# Autodesk Inventor assembly: EFOI-10
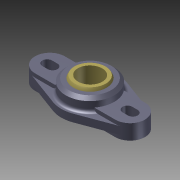
[picture p0: Inventor's stored thumbnail of the model, 180x180]
Saved by Autodesk Inventor 2011 (Build 150239000, 239)
## iProperties
Category: Plastic Bearings
Created: 2008-11-25
Part Number: EFOI-10
Document SubType Name: Assembly
Project: FIRST
Catalog Web Link: http://www.igus.com/pdf/igubal_flange.pdf
Description: Flanged spherical bearing
Vendor: igus
Title: Flanged Spherical Bearing
Author: Autodesk, Inc.
## Documents named in this file (3)
- R:\2012\Inventor\vkop\All-Plastic-Bearings\Plastic Bearings_igus_EFOI-10.iam
- R:\2012\Inventor\vkop\All-Plastic-Bearings\EFOI-10_Housing.ipt
- R:\2012\Inventor\vkop\All-Plastic-Bearings\EFOI-10_Spherical Bearing.ipt
## Components (2 placed, 2 different names)
1. EFOI-10_Housing:1 — Mate:1
2. EFOI-10_Spherical Bearing:1 — Mate:1
## Relationships (1: Mate 1)
- Mate:1: EFOI-10_Housing:1 ↔ EFOI-10_Spherical Bearing:1
